# Autodesk Inventor assembly: BG_Ruder
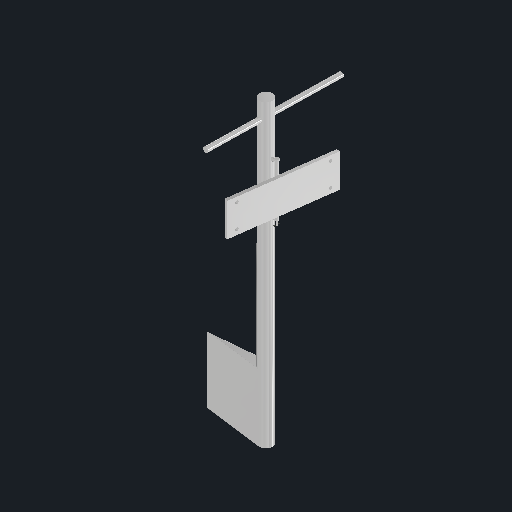
[picture p0: Inventor's stored thumbnail of the model, 512x512]
Saved by Autodesk Inventor 2026.3 (Build 303398000, 398)
## iProperties
Created: 2026-01-29
Part Number: BG_Ruder
Document SubType Name: Assembly
Designer: windows-desktop
Mass: 2105.36 g
Surface Area: 2859.23 cm^2
Volume: 2104.75 cm^3
Density: 1.00029 g/cm^3
Author: windows-desktop
## Documents named in this file (7)
- C:\Users\bluhm\Desktop\Tretboot\Ruder\BG_Ruder.iam
- C:\Users\bluhm\Desktop\Tretboot\Ruder\Bolzen_fuer_Ruder.ipt
- C:\Users\bluhm\Desktop\Tretboot\Ruder\Plattform_mit_Rohr_für_Montierung.ipt
- C:\Users\bluhm\Desktop\Tretboot\Ruder\Ruder_passende_Maße.ipt
- C:\Users\bluhm\Desktop\Tretboot\Ruder\Öse.ipt
- C:\Users\bluhm\Desktop\Tretboot\Normteile\ISO 1234(1)\ISO 1234 - 2,5 x 12DIN EN.ipt
- C:\Users\bluhm\Desktop\Tretboot\Ruder\Lenkstange.ipt
## Components (7 placed, 6 different names)
1. Bolzen_fuer_Ruder:1 — Einfügen:4, Passend:2
2. Plattform_mit_Rohr_für_Montierung:1 — Einfügen:3, Passend:1
3. Ruder_passende_Maße:1 — Einfügen:1, Einfügen:2, Winkel:1, Passend:3
4. Öse:1 — Einfügen:2, Passend:1, Einfügen:4
5. Öse:2 — Einfügen:1, Einfügen:3
6. DIN EN ISO 1234 2,5 x 12:1 — Passend:2
7. Lenkstange:1 — Winkel:1, Passend:3
## Relationships (8: Insert 4, Mate 3, Angle 1)
- Einfügen:1 [Insert]: Ruder_passende_Maße:1 ↔ Öse:2
- Einfügen:2 [Insert]: Ruder_passende_Maße:1 ↔ Öse:1
- Einfügen:3 [Insert]: Plattform_mit_Rohr_für_Montierung:1 ↔ Öse:2
- Passend:1 [Mate]: Plattform_mit_Rohr_für_Montierung:1 ↔ Öse:1
- Einfügen:4 [Insert]: Bolzen_fuer_Ruder:1 ↔ Öse:1
- Passend:2 [Mate]: Bolzen_fuer_Ruder:1 ↔ DIN EN ISO 1234 2,5 x 12:1
- Winkel:1 [Angle] (90 deg): Ruder_passende_Maße:1 ↔ Lenkstange:1
- Passend:3 [Mate]: Ruder_passende_Maße:1 ↔ Lenkstange:1
